# Autodesk Inventor assembly: LightRail_assembly
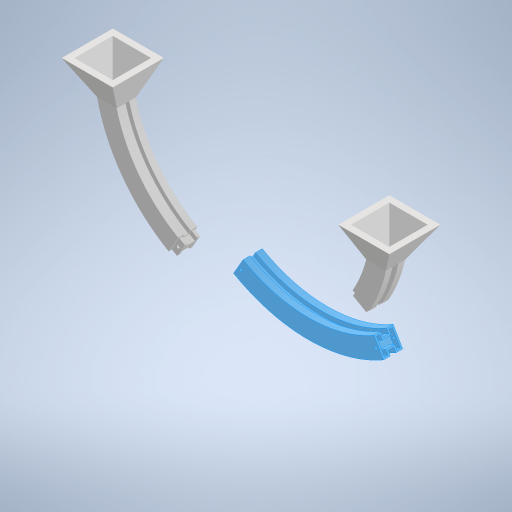
[picture p0: Inventor's stored thumbnail of the model, 512x512]
Saved by Autodesk Inventor 2023 (Build 270158000, 158)
## iProperties
Created: 2023-04-29
Part Number: LightRail_assembly
Document SubType Name: Assembly
Designer: ringl
Author: ringl
## Documents named in this file (4)
- C:\Users\ringl\Documents\Uni Classes\Y3S2\EE318-Project\EE318-Project\CAD\LightRail\LightRail_assembly.iam
- C:\Users\ringl\Documents\Uni Classes\Y3S2\EE318-Project\EE318-Project\CAD\LightRail\LightRail_endSection.ipt
- C:\Users\ringl\Documents\Uni Classes\Y3S2\EE318-Project\EE318-Project\CAD\LightRail\LightRail_middleSection.ipt
- C:\Users\ringl\Documents\Uni Classes\Y3S2\EE318-Project\EE318-Project\CAD\LightRail\LightRail_endMiddleSection.ipt
## Components (4 placed, 3 different names)
1. LightRail_endSection:1 — Flush:1, Mate:1, Mate:2
2. LightRail_middleSection:1
3. LightRail_endSection:2
4. LightRail_endMiddleSection:1 — Flush:1, Mate:1, Mate:2
## Relationships (3: Mate 2, Flush 1)
- Flush:1: LightRail_endSection:1 ↔ LightRail_endMiddleSection:1
- Mate:1: LightRail_endSection:1 ↔ LightRail_endMiddleSection:1
- Mate:2: LightRail_endSection:1 ↔ LightRail_endMiddleSection:1
